# Autodesk Inventor assembly: e3d titan
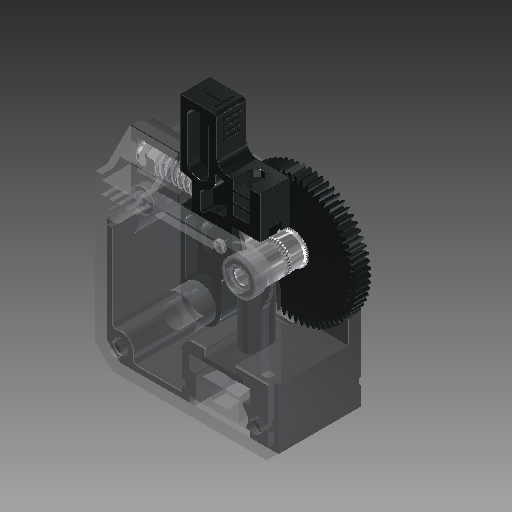
[picture p0: Inventor's stored thumbnail of the model, 512x512]
Saved by Autodesk Inventor 2018 (Build 220112000, 112)
## iProperties
Created: 2016-06-23
Part Number: e3d titan
Document SubType Name: Assembly
Designer: Ben
Author: Ben
## Documents named in this file (14)
- C:\Users\Jurjen\Documents\3D Printer\Own Design\CoreXY\extruder\e3d titan.iam
- C:\Users\Jurjen\Documents\3D Printer\Own Design\CoreXY\extruder\Base.ipt
- C:\Users\Jurjen\Documents\3D Printer\Own Design\CoreXY\extruder\9x5x3mm bearing.ipt
- C:\Users\Jurjen\Documents\3D Printer\Own Design\CoreXY\extruder\hobbed wheel.ipt
- C:\Users\Jurjen\Documents\3D Printer\Own Design\CoreXY\extruder\filament gear.ipt
- C:\Users\Jurjen\Documents\3D Printer\Own Design\CoreXY\extruder\motor gear.ipt
- C:\Users\Jurjen\Documents\3D Printer\Own Design\CoreXY\extruder\cover.ipt
- C:\Users\Jurjen\Documents\3D Printer\Own Design\CoreXY\extruder\m3x8.ipt
- C:\Users\Jurjen\Documents\3D Printer\Own Design\CoreXY\extruder\M3 nut.ipt
- C:\Users\Jurjen\Documents\3D Printer\Own Design\CoreXY\extruder\idler spring.ipt
- C:\Users\Jurjen\Documents\3D Printer\Own Design\CoreXY\extruder\tensioner.ipt
- C:\Users\Jurjen\Documents\3D Printer\Own Design\CoreXY\extruder\idler bearing pin.ipt
- C:\Users\Jurjen\Documents\3D Printer\Own Design\CoreXY\extruder\idler bearing.ipt
- C:\Users\Jurjen\Documents\3D Printer\Own Design\CoreXY\extruder\guide tube.ipt
## Components (14 placed, 13 different names)
1. Base:1 — Flush:1, Flush:2, Flush:3, Mate:1, Mate:2, Mate:12, Mate:14, Flush:4, Mate:15, Mate:19, Mate:29, Mate:30, Angle:1, Mate:31, Angle:2
2. 9x5x3mm bearing:1 — Mate:1, Mate:2, Mate:3, Mate:4
3. hobbed wheel:1 — Mate:3, Mate:4, Mate:5, Mate:6, Mate:13
4. filament gear:1 — Mate:5, Mate:6, Mate:11, Mate:9, Mate:10, Mate:13
5. motor gear:1 — Mate:11, Mate:9, Mate:10, Mate:12
6. cover:1 — Mate:14, Flush:4, Mate:15, Mate:16, Mate:17, Mate:24
7. 9x5x3mm bearing:2 — Mate:16, Mate:17
8. m3x8:1 — Mate:19, Mate:20, Mate:22, Mate:25, Mate:31
9. M3 nut:1 — Mate:20, Mate:23, Angle:2
10. idler spring:1 — Mate:22, Mate:23, Mate:32
11. tensioner:1 — Mate:24, Mate:25, Mate:26, Mate:28, Mate:32, Flush:5
12. idler bearing pin:1 — Mate:26, Mate:27, Flush:5
13. idler bearing:1 — Mate:27, Mate:28
14. guide tube:1 — Mate:29, Mate:30, Angle:1
## Relationships (35: Mate 28, Flush 5, Angle 2)
- Flush:1: Base:1
- Flush:2: Base:1
- Flush:3: Base:1
- Mate:1: Base:1 ↔ 9x5x3mm bearing:1
- Mate:2: Base:1 ↔ 9x5x3mm bearing:1
- Mate:3: 9x5x3mm bearing:1 ↔ hobbed wheel:1
- Mate:4: 9x5x3mm bearing:1 ↔ hobbed wheel:1
- Mate:5: hobbed wheel:1 ↔ filament gear:1
- Mate:6: hobbed wheel:1 ↔ filament gear:1
- Mate:11 (-2.5 mm): filament gear:1 ↔ motor gear:1
- Mate:9 (21.9203 mm): filament gear:1 ↔ motor gear:1
- Mate:10 (21.9203 mm): filament gear:1 ↔ motor gear:1
- Mate:12: Base:1 ↔ motor gear:1
- Mate:13: hobbed wheel:1 ↔ filament gear:1
- Mate:14: Base:1 ↔ cover:1
- Flush:4: Base:1 ↔ cover:1
- Mate:15: Base:1 ↔ cover:1
- Mate:16: cover:1 ↔ 9x5x3mm bearing:2
- Mate:17: cover:1 ↔ 9x5x3mm bearing:2
- Mate:19: Base:1 ↔ m3x8:1
- Mate:20: m3x8:1 ↔ M3 nut:1
- Mate:22: m3x8:1 ↔ idler spring:1
- Mate:23: M3 nut:1 ↔ idler spring:1
- Mate:24: cover:1 ↔ tensioner:1
- Mate:25: m3x8:1 ↔ tensioner:1
- Mate:26: tensioner:1 ↔ idler bearing pin:1
- Mate:27: idler bearing pin:1 ↔ idler bearing:1
- Mate:28: tensioner:1 ↔ idler bearing:1
- Mate:29: Base:1 ↔ guide tube:1
- Mate:30: Base:1 ↔ guide tube:1
- Angle:1 (180 deg): Base:1 ↔ guide tube:1
- Mate:31: Base:1 ↔ m3x8:1
- Mate:32: idler spring:1 ↔ tensioner:1
- Angle:2 (0 deg): Base:1 ↔ M3 nut:1
- Flush:5: tensioner:1 ↔ idler bearing pin:1
